# Autodesk Inventor assembly: Tower Assembly
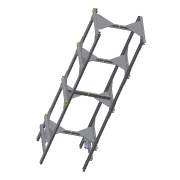
[picture p0: Inventor's stored thumbnail of the model, 180x180]
Saved by Autodesk Inventor 2015 (Build 190159000, 159)
## iProperties
Created: 2015-01-24
Part Number: Tower Assembly
Document SubType Name: Assembly
Designer: Peter
Author: Peter
## Documents named in this file (8)
- T:\FILES\FIRST-Team-1719-CAD-Team\2015 Robot CAD\Two Lifters and Lifter Super Structure\Lifter Super Structure\Tower\Tower Assembly.iam
- T:\FILES\FIRST-Team-1719-CAD-Team\2015 Robot CAD\Two Lifters and Lifter Super Structure\Lifter Super Structure\Tower\Side-Towers Assemblies\Left Side Tower Assembly.iam
- T:\FILES\FIRST-Team-1719-CAD-Team\2015 Robot CAD\Two Lifters and Lifter Super Structure\Lifter Super Structure\Tower\Side-Towers Assemblies\Right Side Tower Assembly.iam
- T:\FILES\FIRST-Team-1719-CAD-Team\2015 Robot CAD\Two Lifters and Lifter Super Structure\Lifter Super Structure\Tower\H-Shaped-Assembly\H-Shaped-Assembly.iam
- T:\FILES\FIRST-Team-1719-CAD-Team\2015 Robot CAD\Two Lifters and Lifter Super Structure\Lifter Super Structure\Tower\Side-Towers Assemblies\Right Side Tower Assembly_MIR.iam
- T:\FILES\FIRST-Team-1719-CAD-Team\2015 Robot CAD\Two Lifters and Lifter Super Structure\Lifter Super Structure\Tower\Side-Towers Assemblies\Left Side Tower Assembly_MIR.iam
- T:\FILES\FIRST-Team-1719-CAD-Team\2015 Robot CAD\Two Lifters and Lifter Super Structure\Lifter Super Structure\Tower\Elevator Motor Assembly\Elevator Motor Assembly.iam
- T:\FILES\FIRST-Team-1719-CAD-Team\2015 Robot CAD\Two Lifters and Lifter Super Structure\Lifter Super Structure\Tower\Elevator Motor Assembly\Elevator Motor Assembly_MIR1.iam
## Components (10 placed, 7 different names)
1. Right Side Tower Assembly:1 [sub-assembly] — Mate:1, Flush:1, Flush:2, Flush:9, Mate:5, Flush:11, Flush:12, Symmetry:1
2. H-Shaped-Assembly:4 [sub-assembly] — Mate:1, Flush:1, Flush:2, Flush:3, Mate:2, Flush:4
3. Left Side Tower Assembly:1 [sub-assembly] — Flush:3, Mate:2, Flush:4, Mate:3, Mate:4, Flush:5, Flush:6, Flush:7, Flush:8, Flush:10, Mate:6
4. H-Shaped-Assembly:5 [sub-assembly] — Mate:3, Flush:5, Flush:8
5. H-Shaped-Assembly:6 [sub-assembly] — Mate:4, Flush:6, Flush:7
6. H-Shaped-Assembly:7 [sub-assembly] — Flush:9, Mate:5, Flush:10
7. Right Side Tower Assembly_MIR:1 [sub-assembly] — Symmetry:1
8. Left Side Tower Assembly_MIR:1 [sub-assembly]
9. Elevator Motor Assembly:1 [sub-assembly] — Mate:6, Flush:11, Flush:12
10. Elevator Motor Assembly_MIR1:1 [sub-assembly]
## Relationships (19: Flush 12, Mate 6, Symmetry 1)
- Mate:1: Right Side Tower Assembly:1 ↔ H-Shaped-Assembly:4
- Flush:1: Right Side Tower Assembly:1 ↔ H-Shaped-Assembly:4
- Flush:2: Right Side Tower Assembly:1 ↔ H-Shaped-Assembly:4
- Flush:3: H-Shaped-Assembly:4 ↔ Left Side Tower Assembly:1
- Mate:2: H-Shaped-Assembly:4 ↔ Left Side Tower Assembly:1
- Flush:4: H-Shaped-Assembly:4 ↔ Left Side Tower Assembly:1
- Mate:3: Left Side Tower Assembly:1 ↔ H-Shaped-Assembly:5
- Mate:4: Left Side Tower Assembly:1 ↔ H-Shaped-Assembly:6
- Flush:5: Left Side Tower Assembly:1 ↔ H-Shaped-Assembly:5
- Flush:6: Left Side Tower Assembly:1 ↔ H-Shaped-Assembly:6
- Flush:7: Left Side Tower Assembly:1 ↔ H-Shaped-Assembly:6
- Flush:8 (-93.6625 mm): Left Side Tower Assembly:1 ↔ H-Shaped-Assembly:5
- Flush:9: Right Side Tower Assembly:1 ↔ H-Shaped-Assembly:7
- Mate:5: Right Side Tower Assembly:1 ↔ H-Shaped-Assembly:7
- Flush:10 (-93.6625 mm): Left Side Tower Assembly:1 ↔ H-Shaped-Assembly:7
- Mate:6: Left Side Tower Assembly:1 ↔ Elevator Motor Assembly:1
- Flush:11: Right Side Tower Assembly:1 ↔ Elevator Motor Assembly:1
- Flush:12 (-165.1 mm): Right Side Tower Assembly:1 ↔ Elevator Motor Assembly:1
- Symmetry:1: Right Side Tower Assembly:1 ↔ Right Side Tower Assembly_MIR:1
## Named parameters: elevator_motor_mount_height = -165.1 mm
